# Autodesk Inventor assembly: BAG_2_Female
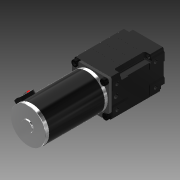
[picture p0: Inventor's stored thumbnail of the model, 180x180]
Saved by Autodesk Inventor 2021 (Build 250183000, 183)
## iProperties
Created: 2018-08-19
Part Number: BAG_2_Female
Document SubType Name: Assembly
Mass: 1123.04 g
Surface Area: 1203.25 cm^2
Volume: 285.054 cm^3
Density: 3.93975 g/cm^3
## Documents named in this file (10)
- D:\FIRST\Design\CollabPartsLib\Motors\FRC\Versaplanetary\VersaPlanetary\BAG, 2 Stages, Female Output.iam
- D:\FIRST\Design\CollabPartsLib\Motors\FRC\Versaplanetary\V2 Stages\V2 Output Stage.iam
- D:\FIRST\Design\CollabPartsLib\Motors\FRC\Versaplanetary\Intermediate Stages\Ring Gear.ipt
- D:\FIRST\Design\CollabPartsLib\Motors\FRC\Versaplanetary\V2 Stages\V2 Input Stage.iam
- D:\FIRST\Design\CollabPartsLib\Motors\FRC\Versaplanetary\Screws\8-32 x 2.25in Screw.ipt
- D:\FIRST\Design\CollabPartsLib\Power Transfer\Bearings\6902ZZ.ipt
- E:\Elipse 6814\Elipse Parts Library\Shaft Accessories\Bearings.ipt
- D:\FIRST\Design\CollabPartsLib\Motors\FRC\Versaplanetary\V2 Stages\V2 Input Stage\VP BAG Input.iam
- D:\FIRST\Design\CollabPartsLib\Motors\FRC\Versaplanetary\VersaPlanetary.iam
- D:\FIRST\Design\CollabPartsLib\Motors\FRC\Versaplanetary\V2 Stages\V2 Output Stage\VP V2 Output Stage Female.iam
## Components (8 placed, 6 different names)
1. VP V2 Output Stage Female:1 [sub-assembly] — Insert:1, Flush:3, Flush:6, 2StageBasicInputMate2, Insert:25
2. Ring Gear 1 — Insert:1, Insert:2, Flush:1, Flush:3
3. Ring Gear 2 — Insert:2, Flush:1, Flush:6, 2StageBasicInputMate1
4. VP BAG Input:1 [sub-assembly] — 2StageBasicInputMate1, 2StageBasicInputMate2, Insert:10, Insert:11
5. 8-32 x 2.25in Screw:1 — Insert:10
6. 8-32 x 2.25in Screw:2 — Insert:11
7. 6902ZZ:1
8. 6902ZZ:2 — Insert:25
## Relationships (10: Insert 6, Flush 4)
- Insert:1: VP V2 Output Stage Female:1 ↔ Ring Gear 1
- Insert:2: Ring Gear 1 ↔ Ring Gear 2
- Flush:1: Ring Gear 1 ↔ Ring Gear 2
- Flush:3: VP V2 Output Stage Female:1 ↔ Ring Gear 1
- Flush:6: VP V2 Output Stage Female:1 ↔ Ring Gear 2
- 2StageBasicInputMate1 [Insert]: Ring Gear 2 ↔ VP BAG Input:1
- 2StageBasicInputMate2 [Flush]: VP V2 Output Stage Female:1 ↔ VP BAG Input:1
- Insert:10: VP BAG Input:1 ↔ 8-32 x 2.25in Screw:1
- Insert:11: VP BAG Input:1 ↔ 8-32 x 2.25in Screw:2
- Insert:25: VP V2 Output Stage Female:1 ↔ 6902ZZ:2
